# Autodesk Inventor assembly: Remote
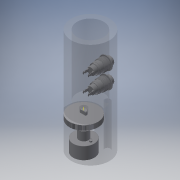
[picture p0: Inventor's stored thumbnail of the model, 180x180]
Saved by Autodesk Inventor 2018 (Build 220112000, 112)
## iProperties
Created: 2019-07-12
Part Number: Remote
Document SubType Name: Assembly
Designer: aal_9
Author: aal_9
## Documents named in this file (5)
- C:\Users\aal_9\OneDrive\Documentos\Suiza\Courses\Tesis\Remote\Remote.iam
- C:\Users\aal_9\OneDrive\Documentos\Suiza\Courses\Tesis\Remote\Housing.ipt
- C:\Users\aal_9\OneDrive\Documentos\Suiza\Courses\Tesis\Remote\PotSensor.ipt
- C:\Users\aal_9\OneDrive\Documentos\Suiza\Courses\Tesis\Remote\Disk.ipt
- C:\Users\aal_9\OneDrive\Documentos\Suiza\Courses\Tesis\Remote\Push_CKCOMPONENTS_8532T1ZBE2\8532T1ZBE2.iam
## Components (5 placed, 4 different names)
1. Housing:1 — Mate:4, Mate:5, Mate:6, Mate:7, Mate:8, Mate:9, Mate:10
2. PotSensor:1 — Mate:1, Mate:2, Mate:3, Mate:4, Mate:5, Mate:6
3. Disk:1 — Mate:1, Mate:2, Mate:3
4. 8532T1ZBE2:1 [sub-assembly] — Mate:7, Mate:10
5. 8532T1ZBE2:2 [sub-assembly] — Mate:8, Mate:9
## Relationships (10: Mate 10)
- Mate:1: PotSensor:1 ↔ Disk:1
- Mate:2: PotSensor:1 ↔ Disk:1
- Mate:3 (3.75 mm): PotSensor:1 ↔ Disk:1
- Mate:4: Housing:1 ↔ PotSensor:1
- Mate:5: Housing:1 ↔ PotSensor:1
- Mate:6: Housing:1 ↔ PotSensor:1
- Mate:7: Housing:1 ↔ 8532T1ZBE2:1
- Mate:8: Housing:1 ↔ 8532T1ZBE2:2
- Mate:9: Housing:1 ↔ 8532T1ZBE2:2
- Mate:10: Housing:1 ↔ 8532T1ZBE2:1
